# Autodesk Inventor assembly: AM14U3+Square+REV1-1
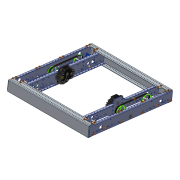
[picture p0: Inventor's stored thumbnail of the model, 180x180]
Saved by Autodesk Inventor 2016 (Build 200138000, 138)
## iProperties
Created: 2015-12-07
Part Number: AM14U3+Square+REV1-1
Description: STEP AP214
Document SubType Name: Assembly
Designer: PrashantBIA
Sending System: SolidWorks 2014
Preprocessor: SwSTEP 2.0
Title: AM14U3 Square REV1-1.STEP
Revision Number: ANY
## Documents named in this file (2)
- C:\Users\PrashantBIA\Desktop\Robotics\Robot Assembly 1-27-15 New Swami\Robot Assembly\Drive Train\AM14U3+Square+REV1-1.iam
- C:\Users\PrashantBIA\Desktop\Robotics\Robot Assembly 1-27-15 New Swami\Robot Assembly\Drive Train\AM14U3 Square Half.iam
## Components (2 placed, 2 different names)
1. AM14U3 Square Half_1 [sub-assembly] — Mate:1, Mate:2
2. AM14U3 Square Half_2 [sub-assembly] — Mate:1, Mate:2
## Relationships (2: Mate 2)
- Mate:1: AM14U3 Square Half_1 ↔ AM14U3 Square Half_2
- Mate:2: AM14U3 Square Half_1 ↔ AM14U3 Square Half_2
